# Autodesk Inventor assembly: Robot Assembly
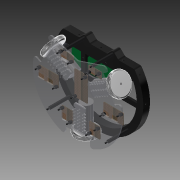
[picture p0: Inventor's stored thumbnail of the model, 180x180]
Saved by Autodesk Inventor 2015 (Build 190159000, 159)
## iProperties
Created: 2016-02-10
Part Number: Robot Assembly
Document SubType Name: Assembly
Designer: James
Mass: 853.796 g
Surface Area: 1762.91 cm^2
Volume: 370.552 cm^3
Density: 2.30412 g/cm^3
Author: James
## Documents named in this file (11)
- C:\Users\James\Dropbox\Robotics 2016\Design\3D Printing\Version 3\Robot Assembly.iam
- C:\Users\James\Dropbox\Robotics 2016\Design\3D Printing\Version 3\Bottom Plate.ipt
- C:\Users\James\Dropbox\Robotics 2016\Design\3D Printing\Motor Mount Standoff.ipt
- C:\Users\James\Dropbox\Robotics 2016\Design\3D Printing\Motor Mount Bracket.ipt
- C:\Users\James\Dropbox\Robotics 2016\Design\3D Printing\Motor.ipt
- C:\Users\James\Dropbox\Robotics 2016\Design\3D Printing\Wheel.ipt
- C:\Users\James\Dropbox\Robotics 2016\Design\3D Printing\Spacer 45.ipt
- C:\Users\James\Dropbox\Robotics 2016\Design\3D Printing\Version 3\Middle Plate.ipt
- C:\Users\James\Dropbox\Robotics 2016\Design\3D Printing\ArduinoMEGA2560.ipt
- C:\Users\James\Dropbox\Robotics 2016\Design\3D Printing\Spacer 5.ipt
- C:\Users\James\Dropbox\Robotics 2016\Design\3D Printing\Version 3\Bottom Plate Veroboard.ipt
## Components (40 placed, 10 different names)
1. Bottom Plate:1 — Mate:1, Mate:2, Mate:3, Mate:4, Mate:5, Mate:6, Mate:7, Mate:8, Mate:9, Mate:31, Mate:32, Mate:33, Mate:34, Mate:35, Mate:36, Mate:37, Mate:38, Mate:57, Mate:58, Mate:59, Mate:60, Mate:61, Mate:62, Mate:63, Mate:64, Mate:65, Mate:66, Mate:67, Mate:68, Mate:69, Mate:70, Mate:71, Mate:72, Mate:73, Mate:74, Mate:75, Mate:76, Mate:77, Mate:78, Mate:79, Mate:80, Mate:81, Mate:82, Mate:83, Mate:84
2. Motor Mount Bracket:1 — Mate:16, Mate:17, Mate:18, Mate:20, Mate:24, Mate:25
3. Motor Mount Standoff:1 — Mate:3, Mate:4, Mate:5, Mate:16, Mate:17, Mate:18
4. Motor:1 — Mate:19, Mate:26, Mate:27, Mate:29, Flush:2
5. Motor Mount Bracket:2 — Mate:13, Mate:14, Mate:15, Mate:21, Mate:22, Mate:23
6. Motor Mount Standoff:2 — Mate:2, Mate:6, Mate:7, Mate:13, Mate:14, Mate:15
7. Motor:2 — Mate:20, Mate:24, Mate:25, Mate:28, Flush:1
8. Motor Mount Bracket:3 — Mate:10, Mate:11, Mate:12, Mate:19, Mate:26, Mate:27
9. Motor Mount Standoff:3 — Mate:1, Mate:8, Mate:9, Mate:10, Mate:11, Mate:12
10. Motor:3 — Mate:21, Mate:22, Mate:23, Mate:30, Flush:3
11. Wheel:1 — Mate:28, Flush:1
12. Wheel:2 — Mate:29, Flush:2
13. Wheel:3 — Mate:30, Flush:3
14. Spacer 45:1 — Mate:33, Mate:38, Mate:40
15. Spacer 45:2 — Mate:32, Mate:37, Mate:41
16. Spacer 45:3 — Mate:31, Mate:36, Mate:39
17. Spacer 45:4 — Mate:34, Mate:35
18. Middle Plate:1 — Mate:39, Mate:40, Mate:41, Mate:42, Mate:43, Mate:44, Mate:45, Mate:46, Mate:47, Mate:48, Mate:49, Mate:50, Mate:51, Mate:52, Mate:53
19. -  -:1 — Mate:54, Mate:55, Mate:56
20. Spacer 5:1 — Mate:42, Mate:43
21. Spacer 5:2 — Mate:48, Mate:53, Mate:55
22. Spacer 5:3 — Mate:46, Mate:47, Mate:56
23. Spacer 5:4 — Mate:49, Mate:52
24. Spacer 5:5 — Mate:50, Mate:51
25. Spacer 5:6 — Mate:44, Mate:45, Mate:54
26. Spacer 5:7 — Mate:61, Mate:63
27. Spacer 5:8 — Mate:65, Mate:66
28. Spacer 5:9 — Mate:67, Mate:68
29. Spacer 5:10 — Mate:62, Mate:64
30. Spacer 5:11 — Mate:75, Mate:76, Mate:86
31. Spacer 5:12 — Mate:73, Mate:74, Mate:85
32. Spacer 5:13 — Mate:69, Mate:70
33. Spacer 5:14 — Mate:71, Mate:72, Mate:87
34. Spacer 5:15 — Mate:78, Mate:84
35. Spacer 5:16 — Mate:77, Mate:83
36. Spacer 5:17 — Mate:57, Mate:58
37. Spacer 5:18 — Mate:59, Mate:60
38. Spacer 5:19 — Mate:80, Mate:81
39. Spacer 5:20 — Mate:79, Mate:82
40. Bottom Plate Veroboard:1 — Mate:85, Mate:86, Mate:87
## Relationships (90: Mate 87, Flush 3)
- Mate:1: Bottom Plate:1 ↔ Motor Mount Standoff:3
- Mate:2: Bottom Plate:1 ↔ Motor Mount Standoff:2
- Mate:3: Bottom Plate:1 ↔ Motor Mount Standoff:1
- Mate:4: Bottom Plate:1 ↔ Motor Mount Standoff:1
- Mate:5: Bottom Plate:1 ↔ Motor Mount Standoff:1
- Mate:6: Bottom Plate:1 ↔ Motor Mount Standoff:2
- Mate:7: Bottom Plate:1 ↔ Motor Mount Standoff:2
- Mate:8: Bottom Plate:1 ↔ Motor Mount Standoff:3
- Mate:9: Bottom Plate:1 ↔ Motor Mount Standoff:3
- Mate:10: Motor Mount Bracket:3 ↔ Motor Mount Standoff:3
- Mate:11: Motor Mount Bracket:3 ↔ Motor Mount Standoff:3
- Mate:12: Motor Mount Bracket:3 ↔ Motor Mount Standoff:3
- Mate:13: Motor Mount Bracket:2 ↔ Motor Mount Standoff:2
- Mate:14: Motor Mount Bracket:2 ↔ Motor Mount Standoff:2
- Mate:15: Motor Mount Bracket:2 ↔ Motor Mount Standoff:2
- Mate:16: Motor Mount Bracket:1 ↔ Motor Mount Standoff:1
- Mate:17: Motor Mount Bracket:1 ↔ Motor Mount Standoff:1
- Mate:18: Motor Mount Bracket:1 ↔ Motor Mount Standoff:1
- Mate:19: Motor:1 ↔ Motor Mount Bracket:3
- Mate:20: Motor Mount Bracket:1 ↔ Motor:2
- Mate:21: Motor Mount Bracket:2 ↔ Motor:3
- Mate:22: Motor Mount Bracket:2 ↔ Motor:3
- Mate:23: Motor Mount Bracket:2 ↔ Motor:3
- Mate:24: Motor Mount Bracket:1 ↔ Motor:2
- Mate:25: Motor Mount Bracket:1 ↔ Motor:2
- Mate:26: Motor:1 ↔ Motor Mount Bracket:3
- Mate:27: Motor:1 ↔ Motor Mount Bracket:3
- Mate:28: Motor:2 ↔ Wheel:1
- Flush:1: Motor:2 ↔ Wheel:1
- Mate:29: Motor:1 ↔ Wheel:2
- Flush:2: Motor:1 ↔ Wheel:2
- Mate:30: Motor:3 ↔ Wheel:3
- Flush:3: Motor:3 ↔ Wheel:3
- Mate:31: Bottom Plate:1 ↔ Spacer 45:3
- Mate:32: Bottom Plate:1 ↔ Spacer 45:2
- Mate:33: Bottom Plate:1 ↔ Spacer 45:1
- Mate:34: Bottom Plate:1 ↔ Spacer 45:4
- Mate:35: Bottom Plate:1 ↔ Spacer 45:4
- Mate:36: Bottom Plate:1 ↔ Spacer 45:3
- Mate:37: Bottom Plate:1 ↔ Spacer 45:2
- Mate:38: Bottom Plate:1 ↔ Spacer 45:1
- Mate:39: Spacer 45:3 ↔ Middle Plate:1
- Mate:40: Spacer 45:1 ↔ Middle Plate:1
- Mate:41: Spacer 45:2 ↔ Middle Plate:1
- Mate:42: Middle Plate:1 ↔ Spacer 5:1
- Mate:43: Middle Plate:1 ↔ Spacer 5:1
- Mate:44: Middle Plate:1 ↔ Spacer 5:6
- Mate:45: Middle Plate:1 ↔ Spacer 5:6
- Mate:46: Middle Plate:1 ↔ Spacer 5:3
- Mate:47: Middle Plate:1 ↔ Spacer 5:3
- Mate:48: Middle Plate:1 ↔ Spacer 5:2
- Mate:49: Middle Plate:1 ↔ Spacer 5:4
- Mate:50: Middle Plate:1 ↔ Spacer 5:5
- Mate:51: Middle Plate:1 ↔ Spacer 5:5
- Mate:52: Middle Plate:1 ↔ Spacer 5:4
- Mate:53: Middle Plate:1 ↔ Spacer 5:2
- Mate:54: -  -:1 ↔ Spacer 5:6
- Mate:55: -  -:1 ↔ Spacer 5:2
- Mate:56: -  -:1 ↔ Spacer 5:3
- Mate:57: Bottom Plate:1 ↔ Spacer 5:17
- Mate:58: Bottom Plate:1 ↔ Spacer 5:17
- Mate:59: Bottom Plate:1 ↔ Spacer 5:18
- Mate:60: Bottom Plate:1 ↔ Spacer 5:18
- Mate:61: Bottom Plate:1 ↔ Spacer 5:7
- Mate:62: Bottom Plate:1 ↔ Spacer 5:10
- Mate:63: Bottom Plate:1 ↔ Spacer 5:7
- Mate:64: Bottom Plate:1 ↔ Spacer 5:10
- Mate:65: Bottom Plate:1 ↔ Spacer 5:8
- Mate:66: Bottom Plate:1 ↔ Spacer 5:8
- Mate:67: Bottom Plate:1 ↔ Spacer 5:9
- Mate:68: Bottom Plate:1 ↔ Spacer 5:9
- Mate:69: Bottom Plate:1 ↔ Spacer 5:13
- Mate:70: Bottom Plate:1 ↔ Spacer 5:13
- Mate:71: Bottom Plate:1 ↔ Spacer 5:14
- Mate:72: Bottom Plate:1 ↔ Spacer 5:14
- Mate:73: Bottom Plate:1 ↔ Spacer 5:12
- Mate:74: Bottom Plate:1 ↔ Spacer 5:12
- Mate:75: Bottom Plate:1 ↔ Spacer 5:11
- Mate:76: Bottom Plate:1 ↔ Spacer 5:11
- Mate:77: Bottom Plate:1 ↔ Spacer 5:16
- Mate:78: Bottom Plate:1 ↔ Spacer 5:15
- Mate:79: Bottom Plate:1 ↔ Spacer 5:20
- Mate:80: Bottom Plate:1 ↔ Spacer 5:19
- Mate:81: Bottom Plate:1 ↔ Spacer 5:19
- Mate:82: Bottom Plate:1 ↔ Spacer 5:20
- Mate:83: Bottom Plate:1 ↔ Spacer 5:16
- Mate:84: Bottom Plate:1 ↔ Spacer 5:15
- Mate:85: Spacer 5:12 ↔ Bottom Plate Veroboard:1
- Mate:86: Spacer 5:11 ↔ Bottom Plate Veroboard:1
- Mate:87: Spacer 5:14 ↔ Bottom Plate Veroboard:1
